# Autodesk Inventor assembly: 組合2
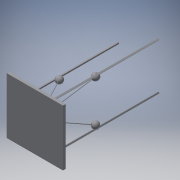
[picture p0: Inventor's stored thumbnail of the model, 180x180]
Saved by Autodesk Inventor 2017 (Build 210142000, 142)
## iProperties
Part Number: 組合2
Material: 一般
Document SubType Name: Assembly
Designer: Brian
Author: Brian
## Documents named in this file (6)
- E:\Brian\001\3D print\組合2.iam
- E:\Brian\001\3D print\底座.ipt
- E:\Brian\001\3D print\軸滑塊.ipt
- E:\Brian\001\3D print\滑桿.ipt
- E:\Brian\001\3D print\噴頭.ipt
- E:\Brian\001\3D print\定位球.ipt
## Components (15 placed, 5 different names)
1. 底座:1 — 貼合:17, 貼合:18, 貼合:19, 貼合:20, 角度:1, 貼合:26, 貼合:27, 角度:2
2. 滑桿:1 — 貼合:21, 貼合:24, 貼合:36
3. 滑桿:2 — 貼合:22, 貼合:23, 貼合:29, 貼合:30
4. 滑桿:3 — 貼合:25, 貼合:28, 貼合:31, 貼合:34
5. 噴頭:1 — 貼合:22, 貼合:24, 角度:1, 貼合:25, 角度:2, 貼合:37
6. 軸滑塊:1 — 貼合:17, 貼合:18, 貼合:23, 齊平:1
7. 軸滑塊:2 — 貼合:19, 貼合:20, 貼合:21, 齊平:2, 貼合:35
8. 軸滑塊:3 — 貼合:26, 貼合:27, 貼合:28, 齊平:1, 齊平:2
9. 定位球:1 — 貼合:34
10. 定位球:4 — 貼合:31
11. 定位球:5 — 貼合:30
12. 定位球:6 — 貼合:29
13. 定位球:7 — 貼合:36
14. 定位球:8 — 貼合:35
15. 定位球:9 — 貼合:37
## Relationships (23: Mate 19, Angle 2, Flush 2)
- 貼合:17 [Mate]: 底座:1 ↔ 軸滑塊:1
- 貼合:18 [Mate]: 底座:1 ↔ 軸滑塊:1
- 貼合:19 [Mate]: 底座:1 ↔ 軸滑塊:2
- 貼合:20 [Mate]: 底座:1 ↔ 軸滑塊:2
- 貼合:21 [Mate]: 滑桿:1 ↔ 軸滑塊:2
- 貼合:22 [Mate]: 滑桿:2 ↔ 噴頭:1
- 貼合:23 [Mate]: 滑桿:2 ↔ 軸滑塊:1
- 貼合:24 [Mate]: 滑桿:1 ↔ 噴頭:1
- 角度:1 [Angle] (0 deg): 底座:1 ↔ 噴頭:1
- 貼合:25 [Mate]: 滑桿:3 ↔ 噴頭:1
- 貼合:26 [Mate]: 底座:1 ↔ 軸滑塊:3
- 貼合:27 [Mate]: 底座:1 ↔ 軸滑塊:3
- 貼合:28 [Mate]: 滑桿:3 ↔ 軸滑塊:3
- 角度:2 [Angle] (0 deg): 底座:1 ↔ 噴頭:1
- 齊平:1 [Flush]: 軸滑塊:1 ↔ 軸滑塊:3
- 齊平:2 [Flush]: 軸滑塊:2 ↔ 軸滑塊:3
- 貼合:29 [Mate]: 滑桿:2 ↔ 定位球:6
- 貼合:30 [Mate]: 滑桿:2 ↔ 定位球:5
- 貼合:31 [Mate]: 滑桿:3 ↔ 定位球:4
- 貼合:34 [Mate]: 滑桿:3 ↔ 定位球:1
- 貼合:35 [Mate]: 軸滑塊:2 ↔ 定位球:8
- 貼合:36 [Mate]: 滑桿:1 ↔ 定位球:7
- 貼合:37 [Mate]: 噴頭:1 ↔ 定位球:9
